# Autodesk Inventor assembly: base4kaki
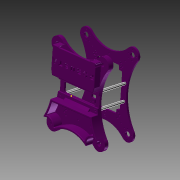
[picture p0: Inventor's stored thumbnail of the model, 180x180]
Saved by Autodesk Inventor 2015 (Build 190159000, 159)
## iProperties
Created: 2015-01-15
Part Number: base4kaki
Document SubType Name: Assembly
Designer: Rafi Kurnia Putra
Author: Rafi Kurnia Putra
## Documents named in this file (7)
- D:\Dropbox\krpai berkaki trui 2015\ROBUSTA\MEKANIK\Grand design\base\base4kaki.iam
- D:\Dropbox\krpai berkaki trui 2015\ROBUSTA\MEKANIK\Grand design\base\BAWAH4.ipt
- D:\Dropbox\krpai berkaki trui 2015\ROBUSTA\MEKANIK\Grand design\base\ATAS4baru.ipt
- D:\Dropbox\krpai berkaki trui 2015\ROBUSTA\MEKANIK\Grand design\base\bawahdepan.ipt
- D:\Dropbox\krpai berkaki trui 2015\ROBUSTA\MEKANIK\Grand design\base\bawahbelakang.ipt
- D:\Dropbox\krpai berkaki trui 2015\ROBUSTA\MEKANIK\Grand design\base\spacer 5 cm.ipt
- D:\Dropbox\krpai berkaki trui 2015\ROBUSTA\MEKANIK\Grand design\base\rumahbearing.ipt
## Components (9 placed, 6 different names)
1. BAWAH4:1 — Mate:10, Mate:11, Mate:12, Mate:13, Mate:14, Mate:15, Rigid:1, Rotational:1, Rotational:2, Rigid:2
2. ATAS4baru:1 — Mate:16, Mate:17, Mate:18
3. bawahdepan:1 — Mate:10, Mate:11, Mate:12
4. bawahbelakang:1 — Mate:13, Mate:14, Mate:15, Mate:19, Mate:20, Angle:1
5. spacer 5 cm:1 — Rigid:1, Mate:18
6. spacer 5 cm:2 — Rotational:2
7. spacer 5 cm:3 — Rigid:2
8. spacer 5 cm:4 — Rotational:1, Mate:16, Mate:17
9. rumahbearing:1 — Mate:19, Mate:20, Angle:1
## Relationships (16: Mate 11, WeldJoint 2, RevoluteJoint 2, Angle 1)
- Mate:10: BAWAH4:1 ↔ bawahdepan:1
- Mate:11: BAWAH4:1 ↔ bawahdepan:1
- Mate:12: BAWAH4:1 ↔ bawahdepan:1
- Mate:13: BAWAH4:1 ↔ bawahbelakang:1
- Mate:14: BAWAH4:1 ↔ bawahbelakang:1
- Mate:15: BAWAH4:1 ↔ bawahbelakang:1
- Rigid:1 [WeldJoint]: BAWAH4:1 ↔ spacer 5 cm:1
- Rotational:1 [RevoluteJoint]: BAWAH4:1 ↔ spacer 5 cm:4
- Rotational:2 [RevoluteJoint]: BAWAH4:1 ↔ spacer 5 cm:2
- Rigid:2 [WeldJoint]: BAWAH4:1 ↔ spacer 5 cm:3
- Mate:16: ATAS4baru:1 ↔ spacer 5 cm:4
- Mate:17: ATAS4baru:1 ↔ spacer 5 cm:4
- Mate:18: ATAS4baru:1 ↔ spacer 5 cm:1
- Mate:19: bawahbelakang:1 ↔ rumahbearing:1
- Mate:20: bawahbelakang:1 ↔ rumahbearing:1
- Angle:1 (180 deg): bawahbelakang:1 ↔ rumahbearing:1
